# Autodesk Inventor assembly: Chalk Applicator
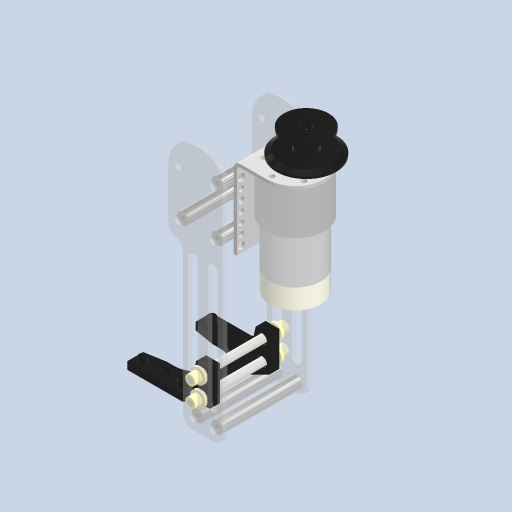
[picture p0: Inventor's stored thumbnail of the model, 512x512]
Saved by Autodesk Inventor 2024 (Build 280153000, 153)
## iProperties
Created: 2023-12-18
Part Number: Chalk Applicator
Document SubType Name: Assembly
Designer: greg
Author: greg
## Documents named in this file (8)
- C:\Users\Greg\Documents\Inventor\Capstone\Chalk Applicator\Chalk Applicator.iam
- C:\Users\Greg\Documents\Inventor\Capstone\Chalk Applicator\Cross Shaft.iam
- C:\Users\Greg\Documents\Inventor\Capstone\Chalk Applicator\Side Plate.ipt
- C:\Users\Greg\Documents\Inventor\Capstone\Chalk Applicator\Standoff.ipt
- C:\Users\greg\Documents\Inventor\Content Center Files\R2024\en-US\ANSI B18.6.3(60)\ANSI B18.6.3 - 6-32 UNC - 1.25(25).ipt
- C:\Users\Greg\Documents\Inventor\Capstone\Chalk Applicator\Vince-Motor.iam
- C:\Users\Greg\Documents\Inventor\Capstone\Chalk Applicator\Pulley.ipt
- C:\Users\Greg\Documents\Inventor\Capstone\Chalk Applicator\Carriage.ipt
## Components (22 placed, 7 different names)
1. Side Plate:1 — Insert:6, Insert:7, Insert:8, Insert:9, Insert:10, Mate:1, Mate:2, Mate:3, Mate:4, Mate:5, Mate:6, Mate:7, Mate:8, Mate:9, Mate:10, Mate:21, Tangent:1, Mate:22, Tangent:2, Mate:27
2. Side Plate:2 — Insert:1, Insert:2, Insert:3, Insert:4, Insert:5, Mate:11, Mate:12, Mate:13, Mate:14, Mate:15, Mate:16, Mate:17, Mate:18, Mate:19, Mate:20, Mate:23, Mate:24
3. Cross Shaft:1 [sub-assembly] — Mate:22, Tangent:2, Mate:23, Mate:29
4. Cross Shaft:2 [sub-assembly] — Mate:21, Tangent:1, Mate:24, Mate:28, Mate:30
5. Standoff:1 — Insert:1, Insert:9
6. Standoff:2 — Insert:2, Insert:10
7. Standoff:3 — Insert:3, Insert:6, Tangent:3
8. Standoff:4 — Insert:4, Insert:8
9. Standoff:5 — Insert:5, Insert:7, Tangent:4, Tangent:5, Tangent:6
10. Square Recessed Pan Head Machine Screw - Type III - Inch (IFI) 6-32 UNC - 1.25:1 — Mate:1, Mate:2
11. Square Recessed Pan Head Machine Screw - Type III - Inch (IFI) 6-32 UNC - 1.25:2 — Mate:3, Mate:4
12. Square Recessed Pan Head Machine Screw - Type III - Inch (IFI) 6-32 UNC - 1.25:3 — Mate:5, Mate:6
13. Square Recessed Pan Head Machine Screw - Type III - Inch (IFI) 6-32 UNC - 1.25:4 — Mate:7, Mate:8
14. Square Recessed Pan Head Machine Screw - Type III - Inch (IFI) 6-32 UNC - 1.25:5 — Mate:9, Mate:10
15. Square Recessed Pan Head Machine Screw - Type III - Inch (IFI) 6-32 UNC - 1.25:6 — Mate:11, Mate:12
16. Square Recessed Pan Head Machine Screw - Type III - Inch (IFI) 6-32 UNC - 1.25:7 — Mate:13, Mate:14
17. Square Recessed Pan Head Machine Screw - Type III - Inch (IFI) 6-32 UNC - 1.25:8 — Mate:15, Mate:16
18. Square Recessed Pan Head Machine Screw - Type III - Inch (IFI) 6-32 UNC - 1.25:9 — Mate:17, Mate:18
19. Square Recessed Pan Head Machine Screw - Type III - Inch (IFI) 6-32 UNC - 1.25:10 — Mate:19, Mate:20
20. Vince-Motor:2 [sub-assembly] — Tangent:3, Tangent:4, Tangent:5, Tangent:6, Mate:25, Mate:26, Mate:27
21. Pulley:1 — Mate:25, Mate:26
22. Carriage:1 — Mate:28, Mate:29, Mate:30
## Relationships (46: Mate 30, Insert 10, Tangent 6)
- Insert:1: Side Plate:2 ↔ Standoff:1
- Insert:2: Side Plate:2 ↔ Standoff:2
- Insert:3: Side Plate:2 ↔ Standoff:3
- Insert:4: Side Plate:2 ↔ Standoff:4
- Insert:5: Side Plate:2 ↔ Standoff:5
- Insert:6: Side Plate:1 ↔ Standoff:3
- Insert:7: Side Plate:1 ↔ Standoff:5
- Insert:8: Side Plate:1 ↔ Standoff:4
- Insert:9: Side Plate:1 ↔ Standoff:1
- Insert:10: Side Plate:1 ↔ Standoff:2
- Mate:1: Side Plate:1 ↔ Square Recessed Pan Head Machine Screw - Type III - Inch (IFI) 6-32 UNC - 1.25:1
- Mate:2: Side Plate:1 ↔ Square Recessed Pan Head Machine Screw - Type III - Inch (IFI) 6-32 UNC - 1.25:1
- Mate:3: Side Plate:1 ↔ Square Recessed Pan Head Machine Screw - Type III - Inch (IFI) 6-32 UNC - 1.25:2
- Mate:4: Side Plate:1 ↔ Square Recessed Pan Head Machine Screw - Type III - Inch (IFI) 6-32 UNC - 1.25:2
- Mate:5: Side Plate:1 ↔ Square Recessed Pan Head Machine Screw - Type III - Inch (IFI) 6-32 UNC - 1.25:3
- Mate:6: Side Plate:1 ↔ Square Recessed Pan Head Machine Screw - Type III - Inch (IFI) 6-32 UNC - 1.25:3
- Mate:7: Side Plate:1 ↔ Square Recessed Pan Head Machine Screw - Type III - Inch (IFI) 6-32 UNC - 1.25:4
- Mate:8: Side Plate:1 ↔ Square Recessed Pan Head Machine Screw - Type III - Inch (IFI) 6-32 UNC - 1.25:4
- Mate:9: Side Plate:1 ↔ Square Recessed Pan Head Machine Screw - Type III - Inch (IFI) 6-32 UNC - 1.25:5
- Mate:10: Side Plate:1 ↔ Square Recessed Pan Head Machine Screw - Type III - Inch (IFI) 6-32 UNC - 1.25:5
- Mate:11: Side Plate:2 ↔ Square Recessed Pan Head Machine Screw - Type III - Inch (IFI) 6-32 UNC - 1.25:6
- Mate:12: Side Plate:2 ↔ Square Recessed Pan Head Machine Screw - Type III - Inch (IFI) 6-32 UNC - 1.25:6
- Mate:13: Side Plate:2 ↔ Square Recessed Pan Head Machine Screw - Type III - Inch (IFI) 6-32 UNC - 1.25:7
- Mate:14: Side Plate:2 ↔ Square Recessed Pan Head Machine Screw - Type III - Inch (IFI) 6-32 UNC - 1.25:7
- Mate:15: Side Plate:2 ↔ Square Recessed Pan Head Machine Screw - Type III - Inch (IFI) 6-32 UNC - 1.25:8
- Mate:16: Side Plate:2 ↔ Square Recessed Pan Head Machine Screw - Type III - Inch (IFI) 6-32 UNC - 1.25:8
- Mate:17: Side Plate:2 ↔ Square Recessed Pan Head Machine Screw - Type III - Inch (IFI) 6-32 UNC - 1.25:9
- Mate:18: Side Plate:2 ↔ Square Recessed Pan Head Machine Screw - Type III - Inch (IFI) 6-32 UNC - 1.25:9
- Mate:19: Side Plate:2 ↔ Square Recessed Pan Head Machine Screw - Type III - Inch (IFI) 6-32 UNC - 1.25:10
- Mate:20: Side Plate:2 ↔ Square Recessed Pan Head Machine Screw - Type III - Inch (IFI) 6-32 UNC - 1.25:10
- Mate:21: Side Plate:1 ↔ Cross Shaft:2
- Tangent:1: Side Plate:1 ↔ Cross Shaft:2
- Mate:22: Side Plate:1 ↔ Cross Shaft:1
- Tangent:2: Side Plate:1 ↔ Cross Shaft:1
- Mate:23: Side Plate:2 ↔ Cross Shaft:1
- Mate:24: Side Plate:2 ↔ Cross Shaft:2
- Tangent:3: Standoff:3 ↔ Vince-Motor:2
- Tangent:4: Standoff:5 ↔ Vince-Motor:2
- Tangent:5: Standoff:5 ↔ Vince-Motor:2
- Tangent:6: Standoff:5 ↔ Vince-Motor:2
- Mate:25: Vince-Motor:2 ↔ Pulley:1
- Mate:26: Vince-Motor:2 ↔ Pulley:1
- Mate:27 (6.6675 mm): Side Plate:1 ↔ Vince-Motor:2
- Mate:28: Cross Shaft:2 ↔ Carriage:1
- Mate:29: Cross Shaft:1 ↔ Carriage:1
- Mate:30 (1.5875 mm): Cross Shaft:2 ↔ Carriage:1
